# Autodesk Inventor assembly: Bearing Flat NScrew Slotted
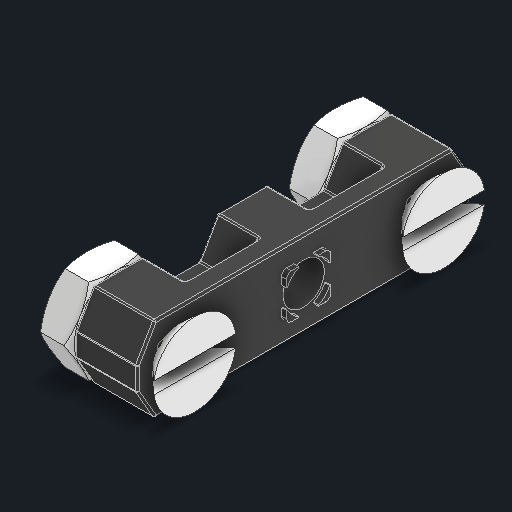
[picture p0: Inventor's stored thumbnail of the model, 512x512]
Saved by Autodesk Inventor 2025.1 (Build 291241000, 241)
## iProperties
Created: 2024-10-10
Part Number: Bearing Flat NScrew Slotted
Document SubType Name: Assembly
Designer: avere
Author: Averey Ku
## Documents named in this file (5)
- C:\Users\avere\VEX\High Stakes\CAD\Codie\Chassis\Drivebay Left\Inner\Bearing Flat NScrew Slotted.iam
- C:\Users\avere\VEX\High Stakes\CAD\Codie\Chassis\Drivebay Left\Inner\NScrew Slotted Threaded .500.ipt
- C:\Users\avere\VEX\High Stakes\CAD\Codie\Chassis\Drivebay Left\Inner\Bearing Flat Low Profile.ipt
- C:\Users\avere\VEX\High Stakes\CAD\ROBOPROS-CAD-Inventor\Structure\Hardware\Nut Nylon\Nut Nylon - White.ipt
- C:\Users\avere\VEX\High Stakes\CAD\ROBOPROS-CAD-Inventor\Structure\Hardware\Nut Nylon.ipt
## Components (7 placed, 3 different names)
1. NScrew Slotted Threaded .500:1 — Insert:1
2. NScrew Slotted Threaded .500:2 — Insert:2
3. Bearing Flat Low Profile:1 — Insert:2, Insert:1, Insert:4, Insert:3, Insert:6, Insert:5
4. Nut Nylon - White:1 — Insert:4
5. Nut Nylon - White:2 — Insert:3
6. NScrew Slotted Threaded .500:3 — Insert:6
7. NScrew Slotted Threaded .500:4 — Insert:5
## Relationships (6: Insert 6)
- Insert:2 (-3.175 mm): NScrew Slotted Threaded .500:2 ↔ Bearing Flat Low Profile:1
- Insert:1 (-3.175 mm): NScrew Slotted Threaded .500:1 ↔ Bearing Flat Low Profile:1
- Insert:4 (1.27 mm): Bearing Flat Low Profile:1 ↔ Nut Nylon - White:1
- Insert:3 (1.27 mm): Bearing Flat Low Profile:1 ↔ Nut Nylon - White:2
- Insert:6 (-1.5875 mm): Bearing Flat Low Profile:1 ↔ NScrew Slotted Threaded .500:3
- Insert:5 (-1.5875 mm): Bearing Flat Low Profile:1 ↔ NScrew Slotted Threaded .500:4
